# Autodesk Inventor assembly: s-assy-shooter_motor
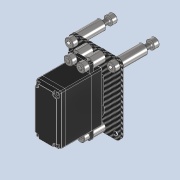
[picture p0: Inventor's stored thumbnail of the model, 180x180]
Saved by Autodesk Inventor 2022 (Build 260153000, 153)
## iProperties
Created: 2021-08-27
Part Number: s-assy-shooter_motor
Document SubType Name: Assembly
Designer: Yuta Kage
Author: Yuta Kage
## Documents named in this file (9)
- C:\Users\yuta0\Desktop\catchrobo_hardware-main\catchrobo_hardware-main\assy-shooter\s-assy-shooter_motor2.iam
- C:\Users\yuta0\Desktop\catchrobo_hardware-main\catchrobo_hardware-main\assy-shooter\MG_996R.iam
- C:\Users\yuta0\Desktop\catchrobo_hardware-main\catchrobo_hardware-main\assy-shooter\ARF-410E.ipt
- C:\Users\yuta0\Desktop\catchrobo_hardware-main\catchrobo_hardware-main\assy-shooter\CB4-6.ipt
- C:\Users\yuta0\Desktop\catchrobo_hardware-main\catchrobo_hardware-main\assy-shooter\CBSTSR4-6.ipt
- C:\Users\yuta0\Desktop\catchrobo_hardware-main\catchrobo_hardware-main\assy-shooter\shooter_carbon_plate4.ipt
- C:\Users\yuta0\Desktop\catchrobo_hardware-main\catchrobo_hardware-main\assy-shooter\CB3-5.ipt
- C:\Users\yuta0\Desktop\catchrobo_hardware-main\catchrobo_hardware-main\assy-shooter\ARF-420E.ipt
- C:\Users\yuta0\Desktop\catchrobo_hardware-main\catchrobo_hardware-main\assy-shooter\CB4-10.ipt
## Components (27 placed, 8 different names)
1. shooter_carbon_plate4:1 — メイト:58, メイト:60, メイト:61, メイト:62, メイト:63, メイト:83, メイト:84, メイト:85, メイト:86
2. MG_996R:1 [sub-assembly] — メイト:22, メイト:56, メイト:57, メイト:61, メイト:64, メイト:65
3. CB3-5:1 — メイト:64, メイト:65
4. ARF-410E:2 — メイト:22, メイト:58, メイト:60
5. CB4-6:9 — メイト:56, メイト:57
6. CBSTSR4-6:1 — メイト:62, メイト:63
7. ARF-410E:3
8. CB4-6:10
9. CBSTSR4-6:2
10. ARF-410E:4
11. CB4-6:11
12. CBSTSR4-6:3
13. ARF-410E:5
14. CB4-6:12
15. CBSTSR4-6:4
16. ARF-420E:1 — メイト:83, メイト:84, メイト:87, メイト:88
17. CB4-6:13 — メイト:85, メイト:86
18. CB4-10:1 — メイト:87, メイト:88
19. ARF-420E:2
20. CB4-6:14
21. CB4-10:2
22. ARF-420E:3
23. CB4-6:15
24. CB4-10:3
25. ARF-420E:4
26. CB4-6:16
27. CB4-10:4
## Component patterns: (4 elements, first: ARF-410E:2 + CB4-6:9 + CBSTSR4-6:1), (4 elements, first: ARF-420E:1 + CB4-6:13 + CB4-10:1)
## Relationships (16: Mate 16)
- メイト:22 [Mate]: MG_996R:1 ↔ ARF-410E:2
- メイト:56 [Mate]: MG_996R:1 ↔ CB4-6:9
- メイト:57 [Mate]: MG_996R:1 ↔ CB4-6:9
- メイト:58 [Mate]: shooter_carbon_plate4:1 ↔ ARF-410E:2
- メイト:60 [Mate]: shooter_carbon_plate4:1 ↔ ARF-410E:2
- メイト:61 [Mate]: shooter_carbon_plate4:1 ↔ MG_996R:1
- メイト:62 [Mate]: shooter_carbon_plate4:1 ↔ CBSTSR4-6:1
- メイト:63 [Mate]: shooter_carbon_plate4:1 ↔ CBSTSR4-6:1
- メイト:64 [Mate]: MG_996R:1 ↔ CB3-5:1
- メイト:65 [Mate]: MG_996R:1 ↔ CB3-5:1
- メイト:83 [Mate]: shooter_carbon_plate4:1 ↔ ARF-420E:1
- メイト:84 [Mate]: shooter_carbon_plate4:1 ↔ ARF-420E:1
- メイト:85 [Mate]: shooter_carbon_plate4:1 ↔ CB4-6:13
- メイト:86 [Mate]: shooter_carbon_plate4:1 ↔ CB4-6:13
- メイト:87 [Mate]: ARF-420E:1 ↔ CB4-10:1
- メイト:88 [Mate] (6 mm): ARF-420E:1 ↔ CB4-10:1
